# Autodesk Inventor assembly: Gobilda Wheel 3606-0001-0096 With Hub
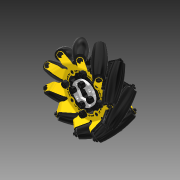
[picture p0: Inventor's stored thumbnail of the model, 180x180]
Saved by Autodesk Inventor 2022 (Build 260153000, 153)
## iProperties
Created: 2021-09-19
Part Number: Gobilda Wheel 3606-0001-0096 With Hub
Document SubType Name: Assembly
## Documents named in this file (7)
- C:\Users\Cal\Desktop\Robotics\Design\Collaborative\Collaborative Parts Library\Wheels and Rollers\Wheels\Gobilda Wheel 3606-0001-0096 With Hub.iam
- C:\Users\Cal\Desktop\Robotics\Design\Collaborative\Collaborative Parts Library\Standard Order Parts\Gobilda Mechanum .5 in Hex Hub (drilled out wheel).ipt
- C:\Users\Cal\Desktop\Robotics\Design\Collaborative\Collaborative Parts Library\Hardware\Nuts\8-32 Pan Head Nylon locknut.ipt
- C:\Users\Cal\Desktop\Robotics\Design\Collaborative\Collaborative Parts Library\Hardware\Nuts.ipt
- C:\Users\Cal\Desktop\Robotics\Design\Collaborative\Collaborative Parts Library\Hardware\Machine Screws\8-32 UNCx0.75 Socket Head Cap Screw.ipt
- C:\Users\Cal\Desktop\Robotics\Design\Collaborative\Collaborative Parts Library\Hardware\Machine Screws.ipt
- C:\Users\Cal\Desktop\Robotics\Design\Collaborative\Collaborative Parts Library\Wheels and Rollers\Wheels\GoBilda Mechanum Wheels 3606-0100-0096.ipt
## Components (11 placed, 4 different names)
1. Gobilda Mechanum .5 in Hex Hub (drilled out wheel):1 — Insert:1, Insert:2
2. Gobilda Mechanum .5 in Hex Hub (drilled out wheel):2 — Insert:3, Insert:4
3. GoBilda Mechanum Wheels 3606-0100-0096:1 — Insert:1, Insert:2, Insert:3, Insert:4
4. 8-32 UNCx0.75 Socket Head Cap Screw:1
5. 8-32 Pan Head Nylon locknut:1
6. 8-32 UNCx0.75 Socket Head Cap Screw:2
7. 8-32 Pan Head Nylon locknut:2
8. 8-32 UNCx0.75 Socket Head Cap Screw:3
9. 8-32 Pan Head Nylon locknut:3
10. 8-32 UNCx0.75 Socket Head Cap Screw:4
11. 8-32 Pan Head Nylon locknut:4
## Component patterns: (4 elements, first: 8-32 UNCx0.75 Socket Head Cap Screw:1 + 8-32 Pan Head Nylon locknut:1)
## Relationships (6: Insert 6)
- Insert:1: Gobilda Mechanum .5 in Hex Hub (drilled out wheel):1 ↔ GoBilda Mechanum Wheels 3606-0100-0096:1
- Insert:2: Gobilda Mechanum .5 in Hex Hub (drilled out wheel):1 ↔ GoBilda Mechanum Wheels 3606-0100-0096:1
- Insert:3: Gobilda Mechanum .5 in Hex Hub (drilled out wheel):2 ↔ GoBilda Mechanum Wheels 3606-0100-0096:1
- Insert:4: Gobilda Mechanum .5 in Hex Hub (drilled out wheel):2 ↔ GoBilda Mechanum Wheels 3606-0100-0096:1
- [Insert]: Gobilda Mechanum .5 in Hex Hub (drilled out wheel):2 ↔ 8-32 Pan Head Nylon locknut:1
- [Insert]: Gobilda Mechanum .5 in Hex Hub (drilled out wheel):1 ↔ 8-32 UNCx0.75 Socket Head Cap Screw:1
